# Autodesk Inventor assembly: Plate Assembly
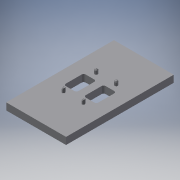
[picture p0: Inventor's stored thumbnail of the model, 180x180]
Saved by Autodesk Inventor 2019.4 (Build 234330000, 330)
## iProperties
Created: 2021-01-14
Part Number: Plate Assembly
Document SubType Name: Assembly
Designer: caleb
Author: caleb
## Documents named in this file (4)
- C:\Users\cfang\Desktop\nebraska-silicon-lab\CAD\TFPX\Wirebonding Plate\Plate Assembly.iam
- C:\Users\cfang\Desktop\nebraska-silicon-lab\CAD\TFPX\Wirebonding Plate\TFPX Plate.ipt
- C:\Users\cfang\Desktop\nebraska-silicon-lab\CAD\TFPX\Wirebonding Plate\8472A190_PRESS-FIT LOCATING PIN.ipt
- C:\Users\cfang\Desktop\nebraska-silicon-lab\CAD\TFPX\Wirebonding Plate\8472A110_PRESS-FIT LOCATING PIN.ipt
## Components (5 placed, 3 different names)
1. TFPX Plate:1 — Insert:1, Insert:2, Insert:3, Insert:4
2. 8472A190_PRESS-FIT LOCATING PIN:1 — Insert:4
3. 8472A110_PRESS-FIT LOCATING PIN:1 — Insert:2
4. 8472A190_PRESS-FIT LOCATING PIN:2 — Insert:3
5. 8472A110_PRESS-FIT LOCATING PIN:2 — Insert:1
## Relationships (4: Insert 4)
- Insert:1: TFPX Plate:1 ↔ 8472A110_PRESS-FIT LOCATING PIN:2
- Insert:2: TFPX Plate:1 ↔ 8472A110_PRESS-FIT LOCATING PIN:1
- Insert:3: TFPX Plate:1 ↔ 8472A190_PRESS-FIT LOCATING PIN:2
- Insert:4: TFPX Plate:1 ↔ 8472A190_PRESS-FIT LOCATING PIN:1
